# Autodesk Inventor assembly: Aero_assembly_skid
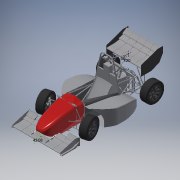
[picture p0: Inventor's stored thumbnail of the model, 180x180]
Saved by Autodesk Inventor 2018 (Build 220112000, 112)
## iProperties
Created: 2018-03-12
Part Number: Aero_assembly_skid
Material: 一般
Document SubType Name: Assembly
Designer: ku_sk
Author: ku_sk
## Documents named in this file (7)
- D:\Users\ku_sk\Documents\Inventor\Aero\KS-15\Aero_assembly_skid.iam
- D:\Users\ku_sk\Documents\Inventor\Aero\KS-15\Fr.wing\Fr.wing_assy.iam
- D:\Users\ku_sk\Documents\Inventor\Aero\KS-15\Rr.wing\Rr.wing_assy.iam
- D:\Users\ku_sk\Documents\Inventor\Aero\KS-15\body\2018 zentai assembly.iam
- D:\Users\ku_sk\Documents\Inventor\Aero\KS-15\Pontoon\2018 radiator analysis.iam
- D:\Users\ku_sk\Documents\Inventor\Aero\KS-15\body\parts\2015Wheel watanabe.ipt
- D:\Users\ku_sk\Documents\Inventor\Aero\KS-15\Fr.wing\cradle\base_model\Fr.wing_cradle(gurnee).ipt
## Components (7 placed, 6 different names)
1. 2018 zentai assembly:1 [sub-assembly] — メイト:8, メイト:9, メイト:10
2. 2018 radiator analysis:1 [sub-assembly] — メイト:11, メイト:12, メイト:13
3. Fr.wing_assy:1 [sub-assembly] — フラッシュ:1, メイト:14, メイト:15, メイト:16
4. Fr.wing_cradle(gurnee):1 — メイト:14, メイト:15, メイト:16
5. Rr.wing_assy:1 [sub-assembly] — フラッシュ:6, フラッシュ:7, フラッシュ:8
6. 2015Wheel watanabe:3 — 角度:2
7. 2015Wheel watanabe:4 — 角度:2
## Relationships (14: Mate 9, Flush 4, Angle 1)
- フラッシュ:1 [Flush]: Fr.wing_assy:1
- フラッシュ:6 [Flush]: Rr.wing_assy:1
- フラッシュ:7 [Flush] (460 mm): Rr.wing_assy:1
- メイト:8 [Mate]: 2018 zentai assembly:1
- メイト:9 [Mate]: 2018 zentai assembly:1
- メイト:10 [Mate]: 2018 zentai assembly:1
- メイト:11 [Mate]: 2018 radiator analysis:1
- メイト:12 [Mate]: 2018 radiator analysis:1
- メイト:13 [Mate]: 2018 radiator analysis:1
- フラッシュ:8 [Flush] (-1080 mm): Rr.wing_assy:1
- 角度:2 [Angle] (0 deg): 2015Wheel watanabe:3 ↔ 2015Wheel watanabe:4
- メイト:14 [Mate]: Fr.wing_assy:1 ↔ Fr.wing_cradle(gurnee):1
- メイト:15 [Mate]: Fr.wing_assy:1 ↔ Fr.wing_cradle(gurnee):1
- メイト:16 [Mate]: Fr.wing_assy:1 ↔ Fr.wing_cradle(gurnee):1
